# Autodesk Inventor assembly: DisplayU_Assembly
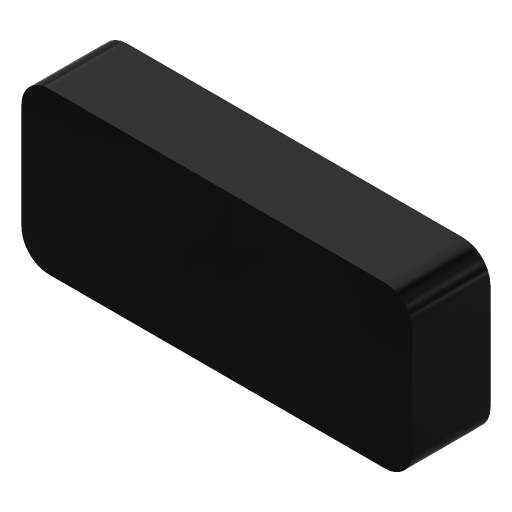
[picture p0: Inventor's stored thumbnail of the model, 512x512]
Saved by Autodesk Inventor 2023.2 (Build 272271000, 271)
## iProperties
Created: 2023-06-14
Part Number: DisplayU_Assembly
Document SubType Name: Assembly
Designer: samdi
Author: samdi
## Documents named in this file (4)
- C:\Users\samdi\Documents\GitHub\embeddedBikeSafety\3D CAD\DisplayU\DisplayU_Assembly.iam
- C:\Users\samdi\Documents\GitHub\embeddedBikeSafety\3D CAD\DisplayU\CASE_0.ipt
- C:\Users\samdi\Documents\GitHub\embeddedBikeSafety\3D CAD\DisplayU\PCB.ipt
- C:\Users\samdi\Documents\GitHub\embeddedBikeSafety\3D CAD\DisplayU\CASE_1.ipt
## Components (3 placed, 3 different names)
1. CASE_0:1 — Mate:1, Flush:1, Flush:2, Mate:2, Mate:3, Mate:4, Flush:3, Flush:4, Mate:5
2. PCB:1 — Mate:2, Mate:3, Mate:4
3. CASE_1:1 — Flush:3, Flush:4, Mate:5
## Relationships (9: Mate 5, Flush 4)
- Mate:1: CASE_0:1
- Flush:1: CASE_0:1
- Flush:2: CASE_0:1
- Mate:2: CASE_0:1 ↔ PCB:1
- Mate:3: CASE_0:1 ↔ PCB:1
- Mate:4: CASE_0:1 ↔ PCB:1
- Flush:3: CASE_0:1 ↔ CASE_1:1
- Flush:4: CASE_0:1 ↔ CASE_1:1
- Mate:5: CASE_0:1 ↔ CASE_1:1
